# Autodesk Inventor assembly: leftside_hinge
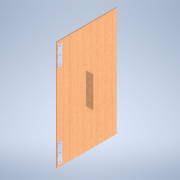
[picture p0: Inventor's stored thumbnail of the model, 180x180]
Saved by Autodesk Inventor 2020 (Build 240168000, 168)
## iProperties
Created: 2020-05-03
Part Number: leftside_hinge
Document SubType Name: Assembly
Designer: galaxy
Author: galaxy
## Documents named in this file (3)
- C:\Users\galaxy\Desktop\control box\leftside_hinge.iam
- C:\Users\galaxy\Desktop\control box\leftside.ipt
- C:\Users\galaxy\Desktop\control box\Peice 1.ipt
## Components (3 placed, 2 different names)
1. leftside:2 — Insert:1, Insert:2, Insert:3, Insert:4
2. Peice 1:1 — Insert:1, Insert:2
3. Peice 1:2 — Insert:3, Insert:4
## Relationships (4: Insert 4)
- Insert:1: leftside:2 ↔ Peice 1:1
- Insert:2: leftside:2 ↔ Peice 1:1
- Insert:3: leftside:2 ↔ Peice 1:2
- Insert:4: leftside:2 ↔ Peice 1:2
